# Autodesk Inventor assembly: Butterfly Drive Base
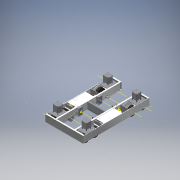
[picture p0: Inventor's stored thumbnail of the model, 180x180]
Saved by Autodesk Inventor 2019 (Build 230136000, 136)
## iProperties
Created: 2019-10-19
Part Number: Butterfly Drive Base
Document SubType Name: Assembly
Designer: Mark
Author: Mark
## Documents named in this file (60)
- C:\Users\Mark\Desktop\7738 Helion Engineering\7738-CAD-prep\Butterfly drive\Butterfly Drive Base.iam
- C:\Users\Mark\Desktop\7738 Helion Engineering\7738-CAD-prep\Butterfly drive\Butterfly Drive Module.iam
- C:\Users\Mark\Desktop\7738 Helion Engineering\7738-CAD-prep\Butterfly drive\Side Extrusion.ipt
- C:\Users\Mark\Desktop\7738 Helion Engineering\7738-CAD-prep\Butterfly drive\Module Plate 1.ipt
- C:\Users\Mark\Desktop\7738 Helion Engineering\7738-CAD-prep\Butterfly drive\Back Extrusion 1.ipt
- C:\Users\Mark\Desktop\7738 Helion Engineering\7738-CAD-prep\Butterfly drive\Bumper Plate.ipt
- C:\Users\Mark\Desktop\7738 Helion Engineering\7738-CAD-prep\Butterfly drive\Side Front Extrusion.ipt
- C:\Users\Mark\Desktop\7738 Helion Engineering\7738-CAD-prep\Butterfly drive\F6800Z 10mm ID Flange.ipt
- C:\Users\Mark\Desktop\7738 Helion Engineering\7738-CAD-prep\2 Stage HD - CIM Sport.iam
- C:\Users\Mark\Desktop\7738 Helion Engineering\7738-CAD-prep\am-0255 2.5inch CIM Motor.ipt
- C:\Users\Mark\Desktop\7738 Helion Engineering\7738-CAD-prep\Butterfly drive\Spacer Extrusion.ipt
- C:\Users\Mark\Desktop\7738 Helion Engineering\7738-CAD-prep\Butterfly drive\Butterfly Drive Base\Design Accelerator\Bevel Gears2.iam
- C:\Users\Mark\Desktop\7738 Helion Engineering\7738-CAD-prep\Butterfly drive\Motor Protection Extrusion.ipt
- C:\Users\Mark\Desktop\7738 Helion Engineering\7738-CAD-prep\Butterfly drive\Butterfly Drive Base\Design Accelerator\Synchronous Belts Transmission3.iam
- C:\Users\Mark\Desktop\7738 Helion Engineering\7738-CAD-prep\transmition Axle Support.ipt
- C:\Users\Mark\Desktop\7738 Helion Engineering\7738-CAD-prep\Butterfly drive\Pneumatic Connector.ipt
- C:\Users\Mark\Desktop\7738 Helion Engineering\7738-CAD-prep\Butterfly drive\SDA 63 50 Full.iam
- C:\Users\Mark\Desktop\7738 Helion Engineering\7738-CAD-prep\Butterfly drive\Front Motor Connector.ipt
- C:\Users\Mark\Desktop\7738 Helion Engineering\7738-CAD-prep\Butterfly drive\Bevel holder.ipt
- C:\Users\Mark\Desktop\7738 Helion Engineering\7738-CAD-prep\Butterfly drive\F10-18M Thrust Bearing.ipt
- C:\Users\Mark\Desktop\7738 Helion Engineering\7738-CAD-prep\Butterfly drive\Motor Protection Extrusion_MIR.ipt
- C:\Users\Mark\Desktop\7738 Helion Engineering\7738-CAD-prep\Butterfly drive\Spacer.ipt
- C:\Users\Mark\Desktop\7738 Helion Engineering\7738-CAD-prep\Butterfly drive\F6004.ipt
- C:\Users\Mark\Desktop\7738 Helion Engineering\7738-CAD-prep\Butterfly drive\F6802.ipt
- C:\Users\Mark\Desktop\7738 Helion Engineering\7738-CAD-prep\Butterfly drive\Butterfly Drive Base\Design Accelerator\Shaft1.iam
- C:\Users\Mark\Desktop\7738 Helion Engineering\7738-CAD-prep\Butterfly drive\Butterfly Drive Module_MIR1.iam
- C:\Users\Mark\Desktop\7738 Helion Engineering\7738-CAD-prep\Butterfly drive\Butterfly Drive Base\Design Accelerator\Synchronous Belts Transmission4.iam
- C:\Users\Mark\Desktop\7738 Helion Engineering\7738-CAD-prep\transmition Axle Support_MIR.ipt
- C:\Users\Mark\Desktop\7738 Helion Engineering\7738-CAD-prep\Butterfly drive\Spacer Extrusion_MIR.ipt
- C:\Users\Mark\Desktop\7738 Helion Engineering\7738-CAD-prep\Butterfly drive\Butterfly Drive Base\Design Accelerator\Shaft2.iam
- C:\Users\Mark\Desktop\7738 Helion Engineering\7738-CAD-prep\Butterfly drive\Butterfly Drive Base\Design Accelerator\Shaft3.iam
- C:\Users\Mark\Desktop\7738 Helion Engineering\7738-CAD-prep\Butterfly drive\Butterfly Drive Module_MIR2.iam
- C:\Users\Mark\Desktop\7738 Helion Engineering\7738-CAD-prep\Butterfly drive\Butterfly Drive Module_MIR1_MIR.iam
- C:\Users\Mark\Desktop\7738 Helion Engineering\7738-CAD-prep\Butterfly drive\Side Extrusion_MIR1.ipt
- C:\Users\Mark\Desktop\7738 Helion Engineering\7738-CAD-prep\Butterfly drive\Bumper Plate_MIR.ipt
- C:\Users\Mark\Desktop\7738 Helion Engineering\7738-CAD-prep\Butterfly drive\Side Front Extrusion_MIR.ipt
- C:\Users\Mark\Desktop\7738 Helion Engineering\7738-CAD-prep\2 Stage HD - CIM Sport_MIR.iam
- C:\Users\Mark\Desktop\7738 Helion Engineering\7738-CAD-prep\am-0255 2.5inch CIM Motor_MIR.ipt
- C:\Users\Mark\Desktop\7738 Helion Engineering\7738-CAD-prep\Butterfly drive\Spacer Extrusion_MIR1.ipt
- C:\Users\Mark\Desktop\7738 Helion Engineering\7738-CAD-prep\Butterfly drive\Butterfly Drive Base\Design Accelerator\Bevel Gears2_MIR.iam
- C:\Users\Mark\Desktop\7738 Helion Engineering\7738-CAD-prep\Butterfly drive\Motor Protection Extrusion_MIR1.ipt
- C:\Users\Mark\Desktop\7738 Helion Engineering\7738-CAD-prep\Butterfly drive\Butterfly Drive Base\Design Accelerator\Synchronous Belts Transmission3_MIR.iam
- C:\Users\Mark\Desktop\7738 Helion Engineering\7738-CAD-prep\transmition Axle Support_MIR1.ipt
- C:\Users\Mark\Desktop\7738 Helion Engineering\7738-CAD-prep\Butterfly drive\Pneumatic Connector_MIR.ipt
- C:\Users\Mark\Desktop\7738 Helion Engineering\7738-CAD-prep\Butterfly drive\SDA 63 50 Full_MIR.iam
- C:\Users\Mark\Desktop\7738 Helion Engineering\7738-CAD-prep\Butterfly drive\Front Motor Connector_MIR.ipt
- C:\Users\Mark\Desktop\7738 Helion Engineering\7738-CAD-prep\Butterfly drive\Bevel holder_MIR.ipt
- C:\Users\Mark\Desktop\7738 Helion Engineering\7738-CAD-prep\Butterfly drive\F10-18M Thrust Bearing_MIR.ipt
- C:\Users\Mark\Desktop\7738 Helion Engineering\7738-CAD-prep\Butterfly drive\Motor Protection Extrusion_MIR_MIR.ipt
- C:\Users\Mark\Desktop\7738 Helion Engineering\7738-CAD-prep\Butterfly drive\F6800Z 10mm ID Flange_MIR1.ipt
- C:\Users\Mark\Desktop\7738 Helion Engineering\7738-CAD-prep\Butterfly drive\Spacer_MIR.ipt
- C:\Users\Mark\Desktop\7738 Helion Engineering\7738-CAD-prep\Butterfly drive\F6004_MIR1.ipt
- C:\Users\Mark\Desktop\7738 Helion Engineering\7738-CAD-prep\Butterfly drive\F6802_MIR1.ipt
- C:\Users\Mark\Desktop\7738 Helion Engineering\7738-CAD-prep\Butterfly drive\Butterfly Drive Base\Design Accelerator\Shaft1_MIR.iam
- C:\Users\Mark\Desktop\7738 Helion Engineering\7738-CAD-prep\Butterfly drive\Butterfly Drive Base\Design Accelerator\Synchronous Belts Transmission4_MIR.iam
- C:\Users\Mark\Desktop\7738 Helion Engineering\7738-CAD-prep\transmition Axle Support_MIR_MIR.ipt
- C:\Users\Mark\Desktop\7738 Helion Engineering\7738-CAD-prep\Butterfly drive\Spacer Extrusion_MIR_MIR.ipt
- C:\Users\Mark\Desktop\7738 Helion Engineering\7738-CAD-prep\Butterfly drive\Butterfly Drive Base\Design Accelerator\Shaft2_MIR.iam
- C:\Users\Mark\Desktop\7738 Helion Engineering\7738-CAD-prep\Butterfly drive\Butterfly Drive Base\Design Accelerator\Shaft3_MIR.iam
- C:\Users\Mark\Desktop\7738 Helion Engineering\7738-CAD-prep\Butterfly drive\Mid support.ipt
## Components (100 placed, 55 different names)
1. Butterfly Drive Module:1 [sub-assembly] — Mate:94, Mate:103, Angle:5, Mate:120
2. Butterfly Drive Module_MIR1:1 [sub-assembly] — Mate:104, Mate:105, Angle:6, Mate:119
3. Back Extrusion 1:1 — Mate:121, Mate:122, Flush:23, Mate:128, Flush:29, Mate:137, Symmetry:2, Mate:227, Flush:64, Mate:228, Mate:230, Mate:233
4. Side Extrusion:1 — Flush:7, Mate:10, Flush:8, Flush:9, Mate:20, Mate:26, Symmetry:1, Angle:2, Flush:11, Flush:15, Angle:3, Mate:47, Flush:18, Flush:19, Mate:63, Mate:69, Mate:70, Rotational:5, Rotational:6, Mate:91, Rotational:9, Mate:93, Mate:94, Angle:5, Mate:104, Mate:105, Angle:6, Mate:106, Flush:22, Flush:23, Flush:26, Mate:126, Mate:128, Mate:129, Flush:27, Mate:131, Rotational:10, Mate:132, Mate:133, Mate:136, Flush:33, Flush:34, Flush:37, Flush:65, Mate:234
5. Bumper Plate:1 — Mate:26, Mate:35, Mate:37, Flush:13, Mate:57, Rotational:7, Mate:122, Flush:24, Flush:25, Rotational:13, Symmetry:2
6. Side Front Extrusion:1 — Flush:7, Mate:10, Flush:8, Symmetry:1, Mate:51, Mate:58, Flush:24, Flush:25, Mate:231
7. 2 Stage HD - CIM Sport:1 [sub-assembly] — Mate:15, Mate:16, Mate:17, Mate:20, Mate:33, Mate:34, Flush:15, Flush:16, Mate:51, Mate:54, Mate:55, Mate:56
8. am-0255 2.5inch CIM Motor:1 — Mate:15, Mate:16, Mate:17, Flush:17
9. 2 Stage HD - CIM Sport:2 [sub-assembly] — Mate:32, Flush:16, Mate:41, Flush:17, Mate:57
10. am-0255 2.5inch CIM Motor:2
11. Spacer Extrusion:2 — Mate:136, Mate:137, Flush:33
12. Bevel Gears:2 [sub-assembly] — Mate:33, Angle:2, Mate:34, Mate:43, Mate:130
13. Bevel Gears:3 [sub-assembly] — Mate:32, Mate:41, Mate:68, Mate:76, Mate:79, Mate:80, Mate:81
14. Spacer Extrusion:3 — Flush:11, Mate:35, Mate:131, Flush:31, Flush:32, Mate:135
15. Motor Protection Extrusion:2 — Mate:37, Flush:13, Mate:62, Mate:64, Mate:65, Flush:20, Flush:21, Mate:231
16. Synchronous Belts Transmission:1 [sub-assembly] — Mate:97, Mate:125, Mate:130, Mate:139
17. transmition Axle Support:1 — Mate:47, Flush:18, Mate:70, Mate:97, Rotational:15
18. Pneumatic Connector:1 — Mate:58, Flush:19, Rigid:1, Mate:69, Mate:82, Mate:83, Mate:84, Mate:85, Mate:86, Mate:87, Mate:88, Mate:89
19. SDA 63 50 Full:1 [sub-assembly] — Rigid:1, Mate:98, Mate:99
20. Front Motor Connector:1 — Mate:62, Mate:63, Mate:64, Mate:90
21. Bevel holder:1 — Mate:65, Mate:76, Mate:78, Flush:20, Rotational:1, Rotational:2
22. F10-18M Thrust Bearing:1 — Mate:80, Mate:81
23. Motor Protection Extrusion_MIR:1 — Flush:21, Mate:90, Mate:91
24. F6800Z 10mm ID Flange:3 — Rotational:1
25. F6800Z 10mm ID Flange:4 — Rotational:2
26. F6800Z 10mm ID Flange:5 — Rotational:15, Flush:35
27. F6800Z 10mm ID Flange:7 — Rotational:5
28. Spacer:1 — Mate:82, Mate:83
29. Spacer:2 — Mate:84, Mate:85
30. Spacer:3 — Mate:88, Mate:89
31. Spacer:4 — Mate:86, Mate:87
32. F6004:1 — Rotational:6
33. F6802:1 — Rotational:7, Rotational:8
34. Shaft:1 [sub-assembly] — Rotational:8, Mate:92, Mate:103
35. F6004:2 — Rotational:9
36. Pneumatic Connector:2 — Mate:106, Flush:22, Mate:115, Mate:116, Mate:117, Mate:121
37. SDA 63 50 Full:2 [sub-assembly] — Mate:107, Mate:108, Mate:109, Mate:110, Mate:111, Mate:112, Mate:113, Mate:114
38. Spacer:5 — Mate:109, Mate:112, Mate:115, Mate:116
39. Spacer:6 — Mate:108, Mate:114, Mate:117
40. Spacer:7 — Mate:107, Mate:111
41. Spacer:8 — Mate:110, Mate:113
42. Synchronous Belts Transmission:2 [sub-assembly] — Mate:126, Mate:127, Mate:129
43. F6004:3 — Rotational:10, Mate:138
44. transmition Axle Support_MIR:1 — Mate:132, Mate:133, Mate:134, Rotational:12, Flush:37
45. F6800Z 10mm ID Flange:9 — Rotational:12, Flush:36, Mate:140
46. Spacer Extrusion_MIR:1 — Flush:31, Flush:32, Mate:135
47. Shaft:2 [sub-assembly] — Flush:34, Mate:138
48. F6802:2 — Rotational:13
49. Shaft:3 [sub-assembly] — Mate:139, Flush:35
50. Shaft:4 [sub-assembly] — Flush:36, Mate:140
51. Butterfly Drive Module_MIR2:1 [sub-assembly] — Mate:141, Angle:9, Mate:194, Mate:216
52. Butterfly Drive Module_MIR1_MIR:1 [sub-assembly] — Angle:10, Mate:199, Mate:200, Mate:217
53. Side Extrusion_MIR1:1 — Mate:141, Mate:144, Flush:41, Mate:145, Flush:42, Flush:43, Flush:44, Mate:147, Symmetry:3, Flush:47, Mate:156, Angle:7, Mate:161, Flush:48, Angle:8, Flush:50, Mate:168, Flush:51, Mate:172, Mate:175, Mate:184, Angle:9, Mate:195, Angle:10, Mate:199, Mate:200, Flush:54, Mate:202, Mate:214, Mate:215, Flush:55, Flush:56, Flush:58, Mate:220, Mate:221, Flush:61, Rotational:19, Rotational:20, Rotational:23, Rotational:24, Mate:227, Flush:64
54. Bumper Plate_MIR:1 — Mate:144, Flush:39, Flush:40, Mate:151, Mate:162, Flush:49, Mate:163, Rotational:21, Rotational:27, Mate:228
55. Side Front Extrusion_MIR:1 — Flush:39, Flush:40, Flush:41, Mate:145, Flush:42, Mate:146, Symmetry:3, Mate:173, Mate:232
56. 2 Stage HD - CIM Sport_MIR:1 [sub-assembly] — Mate:146, Flush:44, Mate:147, Mate:148, Mate:149, Mate:150, Flush:46, Mate:157, Mate:158, Mate:169, Mate:170, Mate:171
57. am-0255 2.5inch CIM Motor_MIR:1 — Mate:148, Mate:149, Mate:150, Flush:45
58. 2 Stage HD - CIM Sport_MIR:2 [sub-assembly] — Mate:151, Flush:45, Flush:46, Mate:152, Mate:153, Mate:154, Mate:159, Mate:160
59. am-0255 2.5inch CIM Motor_MIR:2 — Mate:152, Mate:153, Mate:154
60. Spacer Extrusion_MIR1:1 — Flush:47, Mate:156
61. Bevel Gears2_MIR:1 [sub-assembly] — Mate:157, Mate:158, Angle:7, Mate:164, Mate:165
62. Bevel Gears2_MIR:2 [sub-assembly] — Mate:159, Mate:160, Mate:177, Mate:179, Mate:181, Mate:182, Mate:183
63. Spacer Extrusion_MIR1:2 — Mate:161, Mate:162, Flush:48, Mate:223, Flush:59, Flush:60
64. Motor Protection Extrusion_MIR1:1 — Flush:49, Mate:163, Mate:174, Mate:176, Flush:52, Mate:178, Flush:53
65. Synchronous Belts Transmission3_MIR:1 [sub-assembly] — Mate:165, Mate:166, Mate:219, Mate:225
66. transmition Axle Support_MIR1:1 — Mate:166, Flush:50, Mate:168, Rotational:18, Mate:229
67. Pneumatic Connector_MIR:1 — Flush:51, Mate:172, Mate:173, Mate:186, Mate:187, Mate:188, Mate:189, Mate:190, Mate:191, Mate:192, Mate:193, Rigid:2
68. SDA 63 50 Full_MIR:1 [sub-assembly] — Mate:197, Mate:198, Rigid:2
69. Front Motor Connector_MIR:1 — Mate:174, Mate:175, Mate:176, Mate:185
70. Bevel holder_MIR:1 — Flush:52, Mate:177, Mate:178, Mate:180, Rotational:16, Rotational:17
71. F10-18M Thrust Bearing_MIR:1 — Mate:182, Mate:183
72. Motor Protection Extrusion_MIR_MIR:1 — Mate:184, Mate:185, Flush:53, Mate:232
73. F6800Z 10mm ID Flange_MIR1:1 — Rotational:16
74. F6800Z 10mm ID Flange_MIR1:2 — Rotational:17
75. F6800Z 10mm ID Flange_MIR1:3 — Flush:62, Rotational:18
76. F6800Z 10mm ID Flange_MIR1:4 — Rotational:19
77. Spacer_MIR:1 — Mate:186, Mate:187
78. Spacer_MIR:2 — Mate:188, Mate:189
79. Spacer_MIR:3 — Mate:190, Mate:191
80. Spacer_MIR:4 — Mate:192, Mate:193
81. F6004_MIR1:1 — Rotational:20
82. F6802_MIR1:1 — Rotational:21, Rotational:22
83. Shaft1_MIR:1 [sub-assembly] — Mate:194, Mate:196, Rotational:22
84. F6004_MIR1:2 — Rotational:23
85. Pneumatic Connector_MIR:2 — Flush:54, Mate:202, Mate:203, Mate:204, Mate:207, Mate:230
86. SDA 63 50 Full_MIR:2 [sub-assembly] — Mate:205, Mate:206, Mate:208, Mate:209, Mate:210, Mate:211, Mate:212, Mate:213
87. Spacer_MIR:5 — Mate:203, Mate:204, Mate:205, Mate:206
88. Spacer_MIR:6 — Mate:207, Mate:208, Mate:209
89. Spacer_MIR:7 — Mate:210, Mate:211
90. Spacer_MIR:8 — Mate:212, Mate:213
91. Synchronous Belts Transmission4_MIR:1 [sub-assembly] — Mate:214, Mate:215, Mate:218
92. F6004_MIR1:3 — Mate:224, Rotational:24
93. transmition Axle Support_MIR_MIR:1 — Flush:58, Mate:220, Mate:221, Mate:222, Rotational:26
94. F6800Z 10mm ID Flange_MIR1:6 — Mate:226, Flush:63, Rotational:26
95. Spacer Extrusion_MIR_MIR:1 — Mate:223, Flush:59, Flush:60
96. Shaft1_MIR:2 [sub-assembly] — Mate:224, Flush:61
97. F6802_MIR1:2 — Rotational:27
98. Shaft2_MIR:1 [sub-assembly] — Flush:62, Mate:225, Mate:229
99. Shaft3_MIR:1 [sub-assembly] — Mate:226, Flush:63
100. Mid support:1 — Mate:233, Flush:65, Mate:234
## Relationships (266: Mate 177, Flush 54, RevoluteJoint 22, Angle 8, Symmetry 3, WeldJoint 2)
- Flush:7: Side Extrusion:1 ↔ Side Front Extrusion:1
- Mate:10: Side Extrusion:1 ↔ Side Front Extrusion:1
- Flush:8: Side Extrusion:1 ↔ Side Front Extrusion:1
- Flush:9 (-18.548 mm): Side Extrusion:1
- Mate:15: 2 Stage HD - CIM Sport:1 ↔ am-0255 2.5inch CIM Motor:1
- Mate:16: 2 Stage HD - CIM Sport:1 ↔ am-0255 2.5inch CIM Motor:1
- Mate:17 (0.6 mm): 2 Stage HD - CIM Sport:1 ↔ am-0255 2.5inch CIM Motor:1
- Mate:20 (0.6 mm): Side Extrusion:1 ↔ 2 Stage HD - CIM Sport:1
- [Mate]: 2 Stage HD - CIM Sport:2 ↔ am-0255 2.5inch CIM Motor:2
- [Mate]: 2 Stage HD - CIM Sport:2 ↔ am-0255 2.5inch CIM Motor:2
- [Mate] (0.6 mm): 2 Stage HD - CIM Sport:2 ↔ am-0255 2.5inch CIM Motor:2
- Mate:26 (125 mm): Side Extrusion:1 ↔ Bumper Plate:1
- Symmetry:1: Side Extrusion:1 ↔ Side Front Extrusion:1
- Mate:32: 2 Stage HD - CIM Sport:2 ↔ Bevel Gears:3
- Mate:33: 2 Stage HD - CIM Sport:1 ↔ Bevel Gears:2
- Angle:2 (180 deg): Side Extrusion:1 ↔ Bevel Gears:2
- Mate:34 (2 mm): 2 Stage HD - CIM Sport:1 ↔ Bevel Gears:2
- Flush:11: Side Extrusion:1 ↔ Spacer Extrusion:3
- Mate:35: Bumper Plate:1 ↔ Spacer Extrusion:3
- Mate:37: Bumper Plate:1 ↔ Motor Protection Extrusion:2
- Flush:13 (3 mm): Bumper Plate:1 ↔ Motor Protection Extrusion:2
- Flush:15 (26.1875 mm): Side Extrusion:1 ↔ 2 Stage HD - CIM Sport:1
- Flush:16: 2 Stage HD - CIM Sport:1 ↔ 2 Stage HD - CIM Sport:2
- Mate:41 (2 mm): 2 Stage HD - CIM Sport:2 ↔ Bevel Gears:3
- Mate:43: Bevel Gears:2
- Angle:3 (0 deg): Side Extrusion:1
- Flush:17: am-0255 2.5inch CIM Motor:1 ↔ 2 Stage HD - CIM Sport:2
- Mate:47: Side Extrusion:1 ↔ transmition Axle Support:1
- Flush:18: Side Extrusion:1 ↔ transmition Axle Support:1
- Mate:51 (374.508 mm): Side Front Extrusion:1 ↔ 2 Stage HD - CIM Sport:1
- Mate:54: 2 Stage HD - CIM Sport:1
- Mate:55: 2 Stage HD - CIM Sport:1
- Mate:56: 2 Stage HD - CIM Sport:1
- Mate:57 (11.375 mm): Bumper Plate:1 ↔ 2 Stage HD - CIM Sport:2
- Mate:58 (25 mm): Side Front Extrusion:1 ↔ Pneumatic Connector:1
- Flush:19 (-3 mm): Side Extrusion:1 ↔ Pneumatic Connector:1
- Rigid:1 [WeldJoint] (-20 mm): Pneumatic Connector:1 ↔ SDA 63 50 Full:1
- Mate:62: Motor Protection Extrusion:2 ↔ Front Motor Connector:1
- Mate:63 (63 mm): Side Extrusion:1 ↔ Front Motor Connector:1
- Mate:64 (70 mm): Motor Protection Extrusion:2 ↔ Front Motor Connector:1
- Mate:65: Motor Protection Extrusion:2 ↔ Bevel holder:1
- Mate:68: Bevel Gears:3
- Mate:69: Side Extrusion:1 ↔ Pneumatic Connector:1
- Mate:70 (295.226 mm): Side Extrusion:1 ↔ transmition Axle Support:1
- Mate:76 (6.9 mm): Bevel Gears:3 ↔ Bevel holder:1
- Mate:78: Bevel holder:1
- Mate:79: Bevel Gears:3
- Flush:20 (-0.924 mm): Motor Protection Extrusion:2 ↔ Bevel holder:1
- Mate:80 (0.2 mm): Bevel Gears:3 ↔ F10-18M Thrust Bearing:1
- Mate:81: Bevel Gears:3 ↔ F10-18M Thrust Bearing:1
- Rotational:1 [RevoluteJoint]: Bevel holder:1 ↔ F6800Z 10mm ID Flange:3
- Rotational:2 [RevoluteJoint]: Bevel holder:1 ↔ F6800Z 10mm ID Flange:4
- Rotational:5 [RevoluteJoint]: Side Extrusion:1 ↔ F6800Z 10mm ID Flange:7
- Mate:82: Pneumatic Connector:1 ↔ Spacer:1
- Mate:83: Pneumatic Connector:1 ↔ Spacer:1
- Mate:84: Pneumatic Connector:1 ↔ Spacer:2
- Mate:85: Pneumatic Connector:1 ↔ Spacer:2
- Mate:86: Pneumatic Connector:1 ↔ Spacer:4
- Mate:87: Pneumatic Connector:1 ↔ Spacer:4
- Mate:88: Pneumatic Connector:1 ↔ Spacer:3
- Mate:89: Pneumatic Connector:1 ↔ Spacer:3
- Rotational:6 [RevoluteJoint]: Side Extrusion:1 ↔ F6004:1
- Flush:21: Motor Protection Extrusion:2 ↔ Motor Protection Extrusion_MIR:1
- Mate:90: Front Motor Connector:1 ↔ Motor Protection Extrusion_MIR:1
- Mate:91: Side Extrusion:1 ↔ Motor Protection Extrusion_MIR:1
- Rotational:7 [RevoluteJoint]: Bumper Plate:1 ↔ F6802:1
- Rotational:8 [RevoluteJoint]: F6802:1 ↔ Shaft:1
- Rotational:9 [RevoluteJoint]: Side Extrusion:1 ↔ F6004:2
- Mate:92: Shaft:1
- Mate:93: Side Extrusion:1
- Mate:97 (3 mm): Synchronous Belts Transmission:1 ↔ transmition Axle Support:1
- Mate:94 (6 mm): Butterfly Drive Module:1 ↔ Side Extrusion:1
- Mate:98: SDA 63 50 Full:1
- Mate:99: SDA 63 50 Full:1
- Mate:100
- Mate:101
- Mate:103: Butterfly Drive Module:1 ↔ Shaft:1
- Angle:5 (0 deg): Butterfly Drive Module:1 ↔ Side Extrusion:1
- Mate:104: Butterfly Drive Module_MIR1:1 ↔ Side Extrusion:1
- Mate:105 (6 mm): Butterfly Drive Module_MIR1:1 ↔ Side Extrusion:1
- Angle:6 (0 deg): Butterfly Drive Module_MIR1:1 ↔ Side Extrusion:1
- Mate:106: Side Extrusion:1 ↔ Pneumatic Connector:2
- Flush:22 (-3 mm): Side Extrusion:1 ↔ Pneumatic Connector:2
- Mate:107: SDA 63 50 Full:2 ↔ Spacer:7
- Mate:108: SDA 63 50 Full:2 ↔ Spacer:6
- Mate:109: SDA 63 50 Full:2 ↔ Spacer:5
- Mate:110: SDA 63 50 Full:2 ↔ Spacer:8
- Mate:111: SDA 63 50 Full:2 ↔ Spacer:7
- Mate:112: SDA 63 50 Full:2 ↔ Spacer:5
- Mate:113: SDA 63 50 Full:2 ↔ Spacer:8
- Mate:114: SDA 63 50 Full:2 ↔ Spacer:6
- Mate:115: Pneumatic Connector:2 ↔ Spacer:5
- Mate:116: Pneumatic Connector:2 ↔ Spacer:5
- Mate:117: Pneumatic Connector:2 ↔ Spacer:6
- Mate:119: Butterfly Drive Module_MIR1:1
- Mate:120: Butterfly Drive Module:1
- Mate:121 (20.849 mm): Back Extrusion 1:1 ↔ Pneumatic Connector:2
- Mate:122: Back Extrusion 1:1 ↔ Bumper Plate:1
- Flush:23: Back Extrusion 1:1 ↔ Side Extrusion:1
- Flush:24: Bumper Plate:1 ↔ Side Front Extrusion:1
- Flush:25: Bumper Plate:1 ↔ Side Front Extrusion:1
- Flush:26 (-18.548 mm): Side Extrusion:1
- Mate:125: Synchronous Belts Transmission:1
- Mate:126: Side Extrusion:1 ↔ Synchronous Belts Transmission:2
- Mate:127: Synchronous Belts Transmission:2
- Mate:128: Back Extrusion 1:1 ↔ Side Extrusion:1
- Mate:129 (5 mm): Side Extrusion:1 ↔ Synchronous Belts Transmission:2
- Mate:130: Bevel Gears:2 ↔ Synchronous Belts Transmission:1
- Flush:27: Side Extrusion:1
- Flush:28
- Flush:29: Back Extrusion 1:1
- Flush:30
- Mate:131: Side Extrusion:1 ↔ Spacer Extrusion:3
- Rotational:10 [RevoluteJoint]: Side Extrusion:1 ↔ F6004:3
- Mate:132: Side Extrusion:1 ↔ transmition Axle Support_MIR:1
- Mate:133: Side Extrusion:1 ↔ transmition Axle Support_MIR:1
- Mate:134: transmition Axle Support_MIR:1
- Rotational:12 [RevoluteJoint]: transmition Axle Support_MIR:1 ↔ F6800Z 10mm ID Flange:9
- Flush:31: Spacer Extrusion:3 ↔ Spacer Extrusion_MIR:1
- Flush:32: Spacer Extrusion:3 ↔ Spacer Extrusion_MIR:1
- Mate:135: Spacer Extrusion:3 ↔ Spacer Extrusion_MIR:1
- Mate:136: Side Extrusion:1 ↔ Spacer Extrusion:2
- Mate:137 (642 mm): Back Extrusion 1:1 ↔ Spacer Extrusion:2
- Flush:33: Side Extrusion:1 ↔ Spacer Extrusion:2
- Flush:34 (-31.1 mm): Side Extrusion:1 ↔ Shaft:2
- Mate:138: F6004:3 ↔ Shaft:2
- Rotational:13 [RevoluteJoint]: Bumper Plate:1 ↔ F6802:2
- Mate:139: Synchronous Belts Transmission:1 ↔ Shaft:3
- Rotational:15 [RevoluteJoint]: transmition Axle Support:1 ↔ F6800Z 10mm ID Flange:5
- Flush:35 (-15 mm): F6800Z 10mm ID Flange:5 ↔ Shaft:3
- Symmetry:2: Back Extrusion 1:1 ↔ Bumper Plate:1
- Flush:36 (-14 mm): F6800Z 10mm ID Flange:9 ↔ Shaft:4
- Flush:37: Side Extrusion:1 ↔ transmition Axle Support_MIR:1
- Mate:140: F6800Z 10mm ID Flange:9 ↔ Shaft:4
- Mate:141 (6 mm): Butterfly Drive Module_MIR2:1 ↔ Side Extrusion_MIR1:1
- Mate:144 (125 mm): Side Extrusion_MIR1:1 ↔ Bumper Plate_MIR:1
- Flush:39: Bumper Plate_MIR:1 ↔ Side Front Extrusion_MIR:1
- Flush:40: Bumper Plate_MIR:1 ↔ Side Front Extrusion_MIR:1
- Flush:41: Side Extrusion_MIR1:1 ↔ Side Front Extrusion_MIR:1
- Mate:145: Side Extrusion_MIR1:1 ↔ Side Front Extrusion_MIR:1
- Flush:42: Side Extrusion_MIR1:1 ↔ Side Front Extrusion_MIR:1
- Flush:43 (-18.548 mm): Side Extrusion_MIR1:1
- Mate:146 (374.508 mm): Side Front Extrusion_MIR:1 ↔ 2 Stage HD - CIM Sport_MIR:1
- Flush:44 (26.1875 mm): Side Extrusion_MIR1:1 ↔ 2 Stage HD - CIM Sport_MIR:1
- Mate:147 (0.6 mm): Side Extrusion_MIR1:1 ↔ 2 Stage HD - CIM Sport_MIR:1
- Mate:148 (0.6 mm): 2 Stage HD - CIM Sport_MIR:1 ↔ am-0255 2.5inch CIM Motor_MIR:1
- Mate:149: 2 Stage HD - CIM Sport_MIR:1 ↔ am-0255 2.5inch CIM Motor_MIR:1
- Mate:150: 2 Stage HD - CIM Sport_MIR:1 ↔ am-0255 2.5inch CIM Motor_MIR:1
- Mate:151 (11.375 mm): Bumper Plate_MIR:1 ↔ 2 Stage HD - CIM Sport_MIR:2
- Flush:45: am-0255 2.5inch CIM Motor_MIR:1 ↔ 2 Stage HD - CIM Sport_MIR:2
- Flush:46: 2 Stage HD - CIM Sport_MIR:1 ↔ 2 Stage HD - CIM Sport_MIR:2
- Mate:152: 2 Stage HD - CIM Sport_MIR:2 ↔ am-0255 2.5inch CIM Motor_MIR:2
- Mate:153: 2 Stage HD - CIM Sport_MIR:2 ↔ am-0255 2.5inch CIM Motor_MIR:2
- Mate:154 (0.6 mm): 2 Stage HD - CIM Sport_MIR:2 ↔ am-0255 2.5inch CIM Motor_MIR:2
- Symmetry:3: Side Extrusion_MIR1:1 ↔ Side Front Extrusion_MIR:1
- Flush:47: Side Extrusion_MIR1:1 ↔ Spacer Extrusion_MIR1:1
- Mate:156: Side Extrusion_MIR1:1 ↔ Spacer Extrusion_MIR1:1
- Mate:157 (2 mm): 2 Stage HD - CIM Sport_MIR:1 ↔ Bevel Gears2_MIR:1
- Mate:158: 2 Stage HD - CIM Sport_MIR:1 ↔ Bevel Gears2_MIR:1
- Mate:159 (2 mm): 2 Stage HD - CIM Sport_MIR:2 ↔ Bevel Gears2_MIR:2
- Mate:160: 2 Stage HD - CIM Sport_MIR:2 ↔ Bevel Gears2_MIR:2
- Angle:7 (-180 deg): Side Extrusion_MIR1:1 ↔ Bevel Gears2_MIR:1
- Mate:161: Side Extrusion_MIR1:1 ↔ Spacer Extrusion_MIR1:2
- Mate:162: Bumper Plate_MIR:1 ↔ Spacer Extrusion_MIR1:2
- Flush:48: Side Extrusion_MIR1:1 ↔ Spacer Extrusion_MIR1:2
- Flush:49 (3 mm): Bumper Plate_MIR:1 ↔ Motor Protection Extrusion_MIR1:1
- Mate:163: Bumper Plate_MIR:1 ↔ Motor Protection Extrusion_MIR1:1
- Mate:164: Bevel Gears2_MIR:1
- Mate:165: Bevel Gears2_MIR:1 ↔ Synchronous Belts Transmission3_MIR:1
- Angle:8 (0 deg): Side Extrusion_MIR1:1
- Mate:166 (3 mm): Synchronous Belts Transmission3_MIR:1 ↔ transmition Axle Support_MIR1:1
- Flush:50: Side Extrusion_MIR1:1 ↔ transmition Axle Support_MIR1:1
- Mate:168: Side Extrusion_MIR1:1 ↔ transmition Axle Support_MIR1:1
- Mate:169: 2 Stage HD - CIM Sport_MIR:1
- Mate:170: 2 Stage HD - CIM Sport_MIR:1
- Mate:171: 2 Stage HD - CIM Sport_MIR:1
- Flush:51 (-3 mm): Side Extrusion_MIR1:1 ↔ Pneumatic Connector_MIR:1
- Mate:172: Side Extrusion_MIR1:1 ↔ Pneumatic Connector_MIR:1
- Mate:173 (25 mm): Side Front Extrusion_MIR:1 ↔ Pneumatic Connector_MIR:1
- Mate:174 (70 mm): Motor Protection Extrusion_MIR1:1 ↔ Front Motor Connector_MIR:1
- Mate:175 (63 mm): Side Extrusion_MIR1:1 ↔ Front Motor Connector_MIR:1
- Mate:176: Motor Protection Extrusion_MIR1:1 ↔ Front Motor Connector_MIR:1
- Flush:52 (-0.924 mm): Motor Protection Extrusion_MIR1:1 ↔ Bevel holder_MIR:1
- Mate:177 (6.9 mm): Bevel Gears2_MIR:2 ↔ Bevel holder_MIR:1
- Mate:178: Motor Protection Extrusion_MIR1:1 ↔ Bevel holder_MIR:1
- Mate:179: Bevel Gears2_MIR:2
- Mate:180: Bevel holder_MIR:1
- Mate:181: Bevel Gears2_MIR:2
- Mate:182: Bevel Gears2_MIR:2 ↔ F10-18M Thrust Bearing_MIR:1
- Mate:183 (0.2 mm): Bevel Gears2_MIR:2 ↔ F10-18M Thrust Bearing_MIR:1
- Mate:184: Side Extrusion_MIR1:1 ↔ Motor Protection Extrusion_MIR_MIR:1
- Mate:185: Front Motor Connector_MIR:1 ↔ Motor Protection Extrusion_MIR_MIR:1
- Flush:53: Motor Protection Extrusion_MIR1:1 ↔ Motor Protection Extrusion_MIR_MIR:1
- Mate:186: Pneumatic Connector_MIR:1 ↔ Spacer_MIR:1
- Mate:187: Pneumatic Connector_MIR:1 ↔ Spacer_MIR:1
- Mate:188: Pneumatic Connector_MIR:1 ↔ Spacer_MIR:2
- Mate:189: Pneumatic Connector_MIR:1 ↔ Spacer_MIR:2
- Mate:190: Pneumatic Connector_MIR:1 ↔ Spacer_MIR:3
- Mate:191: Pneumatic Connector_MIR:1 ↔ Spacer_MIR:3
- Mate:192: Pneumatic Connector_MIR:1 ↔ Spacer_MIR:4
- Mate:193: Pneumatic Connector_MIR:1 ↔ Spacer_MIR:4
- Angle:9 (0 deg): Butterfly Drive Module_MIR2:1 ↔ Side Extrusion_MIR1:1
- Mate:194: Butterfly Drive Module_MIR2:1 ↔ Shaft1_MIR:1
- Mate:195: Side Extrusion_MIR1:1
- Mate:196: Shaft1_MIR:1
- Mate:197: SDA 63 50 Full_MIR:1
- Mate:198: SDA 63 50 Full_MIR:1
- Angle:10 (0 deg): Butterfly Drive Module_MIR1_MIR:1 ↔ Side Extrusion_MIR1:1
- Mate:199 (6 mm): Butterfly Drive Module_MIR1_MIR:1 ↔ Side Extrusion_MIR1:1
- Mate:200: Butterfly Drive Module_MIR1_MIR:1 ↔ Side Extrusion_MIR1:1
- Flush:54 (-3 mm): Side Extrusion_MIR1:1 ↔ Pneumatic Connector_MIR:2
- Mate:202: Side Extrusion_MIR1:1 ↔ Pneumatic Connector_MIR:2
- Mate:203: Pneumatic Connector_MIR:2 ↔ Spacer_MIR:5
- Mate:204: Pneumatic Connector_MIR:2 ↔ Spacer_MIR:5
- Mate:205: SDA 63 50 Full_MIR:2 ↔ Spacer_MIR:5
- Mate:206: SDA 63 50 Full_MIR:2 ↔ Spacer_MIR:5
- Mate:207: Pneumatic Connector_MIR:2 ↔ Spacer_MIR:6
- Mate:208: SDA 63 50 Full_MIR:2 ↔ Spacer_MIR:6
- Mate:209: SDA 63 50 Full_MIR:2 ↔ Spacer_MIR:6
- Mate:210: SDA 63 50 Full_MIR:2 ↔ Spacer_MIR:7
- Mate:211: SDA 63 50 Full_MIR:2 ↔ Spacer_MIR:7
- Mate:212: SDA 63 50 Full_MIR:2 ↔ Spacer_MIR:8
- Mate:213: SDA 63 50 Full_MIR:2 ↔ Spacer_MIR:8
- Mate:214 (5 mm): Side Extrusion_MIR1:1 ↔ Synchronous Belts Transmission4_MIR:1
- Mate:215: Side Extrusion_MIR1:1 ↔ Synchronous Belts Transmission4_MIR:1
- Mate:216: Butterfly Drive Module_MIR2:1
- Mate:217: Butterfly Drive Module_MIR1_MIR:1
- Mate:218: Synchronous Belts Transmission4_MIR:1
- Mate:219: Synchronous Belts Transmission3_MIR:1
- Flush:55 (-18.548 mm): Side Extrusion_MIR1:1
- Flush:56: Side Extrusion_MIR1:1
- Flush:58: Side Extrusion_MIR1:1 ↔ transmition Axle Support_MIR_MIR:1
- Mate:220: Side Extrusion_MIR1:1 ↔ transmition Axle Support_MIR_MIR:1
- Mate:221: Side Extrusion_MIR1:1 ↔ transmition Axle Support_MIR_MIR:1
- Mate:222: transmition Axle Support_MIR_MIR:1
- Mate:223: Spacer Extrusion_MIR1:2 ↔ Spacer Extrusion_MIR_MIR:1
- Flush:59: Spacer Extrusion_MIR1:2 ↔ Spacer Extrusion_MIR_MIR:1
- Flush:60: Spacer Extrusion_MIR1:2 ↔ Spacer Extrusion_MIR_MIR:1
- Mate:224: F6004_MIR1:3 ↔ Shaft1_MIR:2
- Flush:61 (-31.1 mm): Side Extrusion_MIR1:1 ↔ Shaft1_MIR:2
- Flush:62 (-15 mm): F6800Z 10mm ID Flange_MIR1:3 ↔ Shaft2_MIR:1
- Mate:225: Synchronous Belts Transmission3_MIR:1 ↔ Shaft2_MIR:1
- Mate:226: F6800Z 10mm ID Flange_MIR1:6 ↔ Shaft3_MIR:1
- Flush:63 (-14 mm): F6800Z 10mm ID Flange_MIR1:6 ↔ Shaft3_MIR:1
- Rigid:2 [WeldJoint] (20 mm): Pneumatic Connector_MIR:1 ↔ SDA 63 50 Full_MIR:1
- Rotational:16 [RevoluteJoint]: Bevel holder_MIR:1 ↔ F6800Z 10mm ID Flange_MIR1:1
- Rotational:17 [RevoluteJoint]: Bevel holder_MIR:1 ↔ F6800Z 10mm ID Flange_MIR1:2
- Rotational:18 [RevoluteJoint]: transmition Axle Support_MIR1:1 ↔ F6800Z 10mm ID Flange_MIR1:3
- Rotational:19 [RevoluteJoint]: Side Extrusion_MIR1:1 ↔ F6800Z 10mm ID Flange_MIR1:4
- Rotational:20 [RevoluteJoint]: Side Extrusion_MIR1:1 ↔ F6004_MIR1:1
- Rotational:21 [RevoluteJoint]: Bumper Plate_MIR:1 ↔ F6802_MIR1:1
- Rotational:22 [RevoluteJoint]: F6802_MIR1:1 ↔ Shaft1_MIR:1
- Rotational:23 [RevoluteJoint]: Side Extrusion_MIR1:1 ↔ F6004_MIR1:2
- Rotational:24 [RevoluteJoint]: Side Extrusion_MIR1:1 ↔ F6004_MIR1:3
- Rotational:26 [RevoluteJoint]: transmition Axle Support_MIR_MIR:1 ↔ F6800Z 10mm ID Flange_MIR1:6
- Rotational:27 [RevoluteJoint]: Bumper Plate_MIR:1 ↔ F6802_MIR1:2
- Mate:227: Back Extrusion 1:1 ↔ Side Extrusion_MIR1:1
- Flush:64: Back Extrusion 1:1 ↔ Side Extrusion_MIR1:1
- Mate:228: Back Extrusion 1:1 ↔ Bumper Plate_MIR:1
- Mate:229: transmition Axle Support_MIR1:1 ↔ Shaft2_MIR:1
- Mate:230 (20.849 mm): Back Extrusion 1:1 ↔ Pneumatic Connector_MIR:2
- Mate:231 (372 mm): Side Front Extrusion:1 ↔ Motor Protection Extrusion:2
- Mate:232 (372 mm): Side Front Extrusion_MIR:1 ↔ Motor Protection Extrusion_MIR_MIR:1
- Mate:233 (450 mm): Back Extrusion 1:1 ↔ Mid support:1
- Flush:65: Side Extrusion:1 ↔ Mid support:1
- Mate:234: Side Extrusion:1 ↔ Mid support:1
## Named parameters: Height = 70 mm, ExtSta = 1 deg, ModuleAngle = 10 deg, d58_d50 = 0.6 mm, d59_d48 = 0 mm, d60_d49 = 0 mm
